# Autodesk Inventor assembly: ASSEMBLY_Tracks
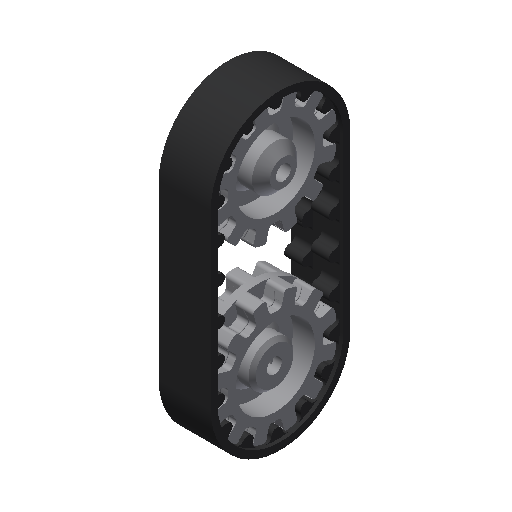
[picture p0: Inventor's stored thumbnail of the model, 512x512]
Saved by Autodesk Inventor 2026.1 (Build 301233000, 233)
## iProperties
Created: 2016-04-29
Part Number: ASSEMBLY_Tracks
Material: Ogólny
Document SubType Name: Assembly
Designer: Andrzej
Mass: 23.1594 g
Surface Area: 178.59 cm^2
Volume: 23.1594 cm^3
Density: 1 g/cm^3
Author: Andrzej
## Documents named in this file (4)
- C:\Users\Andrzej\OneDrive\_DRIVE_SYNCH_FILES\__ BYTECHLAB PROJECTS\MLTDIS - Mini Sumo Robot - Bullet XT\MCAD\1_REV1\ASSEMBLY_MAIN_REVA\ASSEMBLY_Tracks.iam
- C:\Users\Andrzej\OneDrive\_DRIVE_SYNCH_FILES\__ BYTECHLAB PROJECTS\MLTDIS - Mini Sumo Robot - Bullet XT\MCAD\1_REV1\ASSEMBLY_MAIN_REVA\3DP_PLA_Motor_wheel.ipt
- C:\Users\Andrzej\OneDrive\_DRIVE_SYNCH_FILES\__ BYTECHLAB PROJECTS\MLTDIS - Mini Sumo Robot - Bullet XT\MCAD\1_REV1\__COTS_PARTS\COTS_POLOLU_22T_Track.ipt
- C:\Users\Andrzej\OneDrive\_DRIVE_SYNCH_FILES\__ BYTECHLAB PROJECTS\MLTDIS - Mini Sumo Robot - Bullet XT\MCAD\1_REV1\ASSEMBLY_MAIN_REVA\3DP_PLA_Screw_wheel.ipt
## Components (3 placed, 3 different names)
1. 3DP_PLA_Motor_wheel:3 — Zestawiający:2, Równoległy:4
2. 3DP_PLA_Screw_wheel:1 — Zestawiający:1, Równoległy:3
3. COTS_POLOLU_22T_Track:1 — Zestawiający:1, Zestawiający:2, Równoległy:3, Równoległy:4
## Relationships (4: Mate 2, Flush 2)
- Zestawiający:1 [Mate]: 3DP_PLA_Screw_wheel:1 ↔ COTS_POLOLU_22T_Track:1
- Zestawiający:2 [Mate]: 3DP_PLA_Motor_wheel:3 ↔ COTS_POLOLU_22T_Track:1
- Równoległy:3 [Flush]: 3DP_PLA_Screw_wheel:1 ↔ COTS_POLOLU_22T_Track:1
- Równoległy:4 [Flush]: 3DP_PLA_Motor_wheel:3 ↔ COTS_POLOLU_22T_Track:1
